# Autodesk Inventor assembly: CL6-100
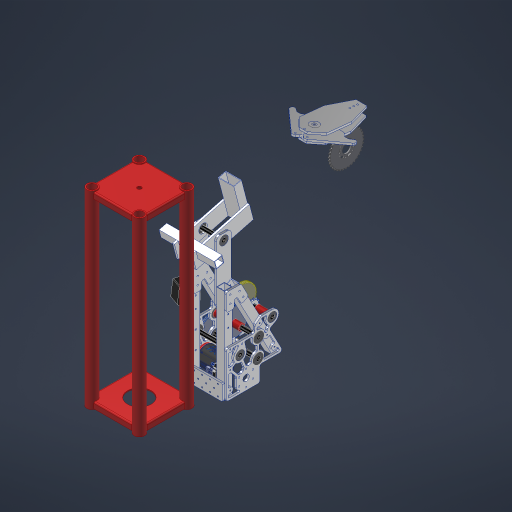
[picture p0: Inventor's stored thumbnail of the model, 512x512]
Saved by Autodesk Inventor 2023.4 (Build 274418000, 418)
## iProperties
Created: 2025-02-04
Part Number: CL6-100
Document SubType Name: Assembly
Designer: brand
Mass: 3247.43 g
Surface Area: 7567.76 cm^2
Volume: 1278.12 cm^3
Author: brand
## Documents named in this file (15)
- C:\Users\brand\OneDrive\Documents\GitHub\robotics 23\2025-ReefScape---CAD\Climber\CL6\CL6-100.iam
- C:\Users\brand\OneDrive\Documents\GitHub\robotics 23\2025-ReefScape---CAD\Climber\CL4\CL4-011.ipt
- C:\Users\brand\OneDrive\Documents\GitHub\robotics 23\2025-ReefScape---CAD\Climber\CL4\CL4-400-GB.iam
- C:\Users\brand\OneDrive\Documents\GitHub\robotics 23\2025-ReefScape---CAD\COMMON PARTS\BEARINGS\0_500_ID_x_1_125_OD_x_0_313_WD_Flanged_Bearing_217-2731.ipt
- C:\Users\brand\OneDrive\Documents\GitHub\robotics 23\2025-ReefScape---CAD\Climber\CL4\CL4-021.ipt
- C:\Users\brand\OneDrive\Documents\GitHub\robotics 23\2025-ReefScape---CAD\COMMON PARTS\ELECTRONICS\cameras\ELP Camera Angled' 17.5 + 7.5 deg up Case.ipt
- C:\Users\brand\OneDrive\Documents\GitHub\robotics 23\2025-ReefScape---CAD\Climber\CL6\CL6-300.iam
- C:\Users\brand\OneDrive\Documents\GitHub\robotics 23\2025-ReefScape---CAD\Field Items\Full Field\FE-2025\GE-25201.iam
- C:\Users\brand\OneDrive\Documents\GitHub\robotics 23\2025-ReefScape---CAD\Climber\CL4\CL4-002.ipt
- C:\Users\brand\OneDrive\Documents\GitHub\robotics 23\2025-ReefScape---CAD\Climber\CL4\CL4-007.ipt
- C:\Users\brand\OneDrive\Documents\GitHub\robotics 23\2025-ReefScape---CAD\Climber\CL4\CL4-009.ipt
- C:\Users\brand\OneDrive\Documents\GitHub\robotics 23\2025-ReefScape---CAD\Climber\CL6\CL6-001.ipt
- C:\Users\brand\OneDrive\Documents\GitHub\robotics 23\2025-ReefScape---CAD\Climber\CL6\CL6-003.ipt
- C:\Users\brand\OneDrive\Documents\GitHub\robotics 23\2025-ReefScape---CAD\Climber\CL6\CL6-004.ipt
- C:\Users\brand\OneDrive\Documents\GitHub\robotics 23\2025-ReefScape---CAD\Climber\CL6\CL6-005.ipt
## Components (20 placed, 14 different names)
1. CL6-300:1 [sub-assembly]
2. CL4-011:1 — Mate:19, Flush:2
3. CL4-400-GB:1 [sub-assembly] — Mate:21
4. 0_500_ID_x_1_125_OD_x_0_313_WD_Flanged_Bearing_217-2731:1
5. 0_500_ID_x_1_125_OD_x_0_313_WD_Flanged_Bearing_217-2731:2 — Mate:19, Flush:2, Mate:24
6. CL4-021:1
7. ELP Camera Angled' 17.5 + 7.5 deg up Case:2
8. GE-25201:1 [sub-assembly] — Mate:21, Mate:23
9. CL4-002:1
10. CL4-002:2
11. CL4-007:1
12. CL4-007:2
13. CL4-009:1
14. CL4-009:2
15. CL6-001:1 — Symmetry:1
16. CL6-001:2 — Symmetry:1, Mate:28
17. CL6-003:1 — Mate:24, Mate:25, Angle:2, Mate:26, Flush:6, Flush:7, Mate:28
18. CL6-004:1 — Mate:26, Flush:6, Flush:7, Mate:27
19. CL6-003:2 — Mate:25, Angle:2, Mate:27, Mate:29, Mate:30
20. CL6-005:1 — Mate:29, Mate:30, Flush:8
## Relationships (39: Insert 19, Mate 11, Flush 6, Angle 2, Symmetry 1)
- [Angle] (0 deg): CL6-300:1 ↔ CL4-002:1
- [Insert]: 0_500_ID_x_1_125_OD_x_0_313_WD_Flanged_Bearing_217-2731:2 ↔ CL6-001:1
- [Insert]: 0_500_ID_x_1_125_OD_x_0_313_WD_Flanged_Bearing_217-2731:1 ↔ CL6-001:2
- Mate:19: CL4-011:1 ↔ 0_500_ID_x_1_125_OD_x_0_313_WD_Flanged_Bearing_217-2731:2
- Flush:2: CL4-011:1 ↔ 0_500_ID_x_1_125_OD_x_0_313_WD_Flanged_Bearing_217-2731:2
- [Insert]: CL4-400-GB:1 ↔ CL4-002:2
- [Insert]: CL4-400-GB:1 ↔ CL4-002:2
- [Insert]: CL4-021:1 ↔ CL4-002:1
- [Insert]: ELP Camera Angled' 17.5 + 7.5 deg up Case:2 ↔ CL4-002:2
- [Insert]: ELP Camera Angled' 17.5 + 7.5 deg up Case:2 ↔ CL4-002:2
- [Insert]: CL4-021:1 ↔ CL4-002:2
- Mate:21 (-80.9752 mm): CL4-400-GB:1 ↔ GE-25201:1
- [Flush]: CL4-002:1 ↔ CL4-002:2
- [Insert]: CL4-007:2 ↔ CL4-009:1
- [Insert]: CL4-007:2 ↔ CL4-009:1
- [Insert]: CL4-002:2 ↔ CL4-009:2
- [Insert]: CL4-002:2 ↔ CL4-009:2
- [Insert]: CL4-007:1 ↔ CL4-009:2
- [Insert]: CL4-007:1 ↔ CL4-009:2
- [Insert]: CL4-007:2 ↔ CL6-001:1
- [Insert]: CL4-002:2 ↔ CL6-001:2
- [Insert]: CL4-007:1 ↔ CL6-001:2
- [Mate] (66.675 mm): CL6-001:1 ↔ CL6-001:2
- [Flush]: CL4-002:1 ↔ CL4-002:2
- [Insert]: CL4-002:1 ↔ CL6-001:1
- [Insert]: CL4-002:1 ↔ CL4-009:1
- Symmetry:1: CL6-001:1 ↔ CL6-001:2
- Mate:23: GE-25201:1
- Mate:24: 0_500_ID_x_1_125_OD_x_0_313_WD_Flanged_Bearing_217-2731:2 ↔ CL6-003:1
- Mate:25: CL6-003:1 ↔ CL6-003:2
- Angle:2 (0 deg): CL6-003:1 ↔ CL6-003:2
- Mate:26: CL6-003:1 ↔ CL6-004:1
- Flush:6: CL6-003:1 ↔ CL6-004:1
- Flush:7: CL6-003:1 ↔ CL6-004:1
- Mate:27: CL6-004:1 ↔ CL6-003:2
- Mate:28: CL6-001:2 ↔ CL6-003:1
- Mate:29: CL6-003:2 ↔ CL6-005:1
- Mate:30: CL6-003:2 ↔ CL6-005:1
- Flush:8: CL6-005:1
